# Autodesk Inventor assembly: ダイクロイックミラー
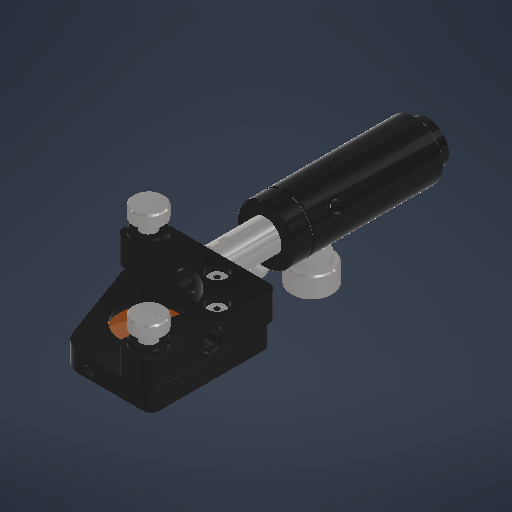
[picture p0: Inventor's stored thumbnail of the model, 512x512]
Saved by Autodesk Inventor 2026 (Build 300175050, 175E)
## iProperties
Created: 2025-07-10
Part Number: ダイクロイックミラー
Document SubType Name: Assembly
Designer: jin20
Author: jin20
## Documents named in this file (5)
- C:\Users\jin20\Documents\装置CAD\RamanSystem\Optics\ダイクロイックミラー.iam
- C:\Users\jin20\Documents\装置CAD\RamanSystem\Optics\ミラーマウント\ミラーマウント.iam
- C:\Users\jin20\Documents\装置CAD\RamanSystem\Optics\ダイクロイックミラー.ipt
- C:\Users\jin20\Documents\装置CAD\RamanSystem\Optics\ロッド\ロッド_60mm.ipt
- C:\Users\jin20\Documents\装置CAD\RamanSystem\Optics\ロッドスタンド.ipt
## Components (4 placed, 4 different names)
1. ミラーマウント:1 [sub-assembly] — 挿入:1, 挿入:2
2. ダイクロイックミラー:1 — 挿入:1
3. ロッド_60mm:1 — 挿入:2, リジッド:1
4. ロッドスタンド:1 — リジッド:1
## Relationships (3: Insert 2, WeldJoint 1)
- 挿入:1 [Insert]: ミラーマウント:1 ↔ ダイクロイックミラー:1
- 挿入:2 [Insert]: ミラーマウント:1 ↔ ロッド_60mm:1
- リジッド:1 [WeldJoint] (20 mm): ロッド_60mm:1 ↔ ロッドスタンド:1
